# Autodesk Inventor assembly: Tamiya SRB u joint
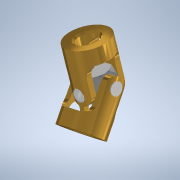
[picture p0: Inventor's stored thumbnail of the model, 180x180]
Saved by Autodesk Inventor 2020 (Build 240168000, 168)
## iProperties
Created: 2015-10-12
Part Number: Tamiya SRB u joint
Document SubType Name: Assembly
Designer: Vikki
Sending System: SolidWorks 2015
Last Author: Tompkins
Last Saved: 2015-10-12
Author: Vikki
## Documents named in this file (12)
- D:\borewell rescuebot\pll manipulator files\sps manipulator\Tamiya SRB u joint.iam
- D:\borewell rescuebot\pll manipulator files\sps manipulator\center block u joint.ipt
- D:\borewell rescuebot\pll manipulator files\sps manipulator\Tamiya u joint.ipt
- D:\borewell rescuebot\pll manipulator files\sps manipulator\large pin.ipt
- D:\borewell rescuebot\pll manipulator files\sps manipulator\small rivit.ipt
- D:\borewell rescuebot\pll manipulator files\sps manipulator\Tamiya u joint - 2.ipt
- D:\borewell rescuebot\pll manipulator files\sps manipulator\Tamiya SRB u joint\AIP\FEA\dh3epo728.fins
- D:\borewell rescuebot\pll manipulator files\sps manipulator\Tamiya SRB u joint\AIP\FEA\dh3epo728.fsat
- D:\borewell rescuebot\pll manipulator files\sps manipulator\Tamiya SRB u joint\AIP\FEA\dh3epo728.ftes
- D:\borewell rescuebot\pll manipulator files\sps manipulator\Tamiya SRB u joint\AIP\FEA\dh3epo728.fwiz
- D:\borewell rescuebot\pll manipulator files\sps manipulator\Tamiya SRB u joint\AIP\FEA\dh3epo734.fmsh
- D:\borewell rescuebot\pll manipulator files\sps manipulator\Tamiya SRB u joint\AIP\FEA\dh3epo735.fres
## Components (5 placed, 5 different names)
1. center block u joint:1 — Mate:3, Mate:4, Mate:7, Mate:11, Mate:12
2. Tamiya u joint:1 — Mate:7, Mate:11, Flush:1
3. large pin:1 — Mate:3, Mate:4, Mate:5, Mate:10
4. small rivit:1 — Mate:5, Flush:1
5. Tamiya u joint - 2:1 — Mate:10, Mate:12
## Relationships (8: Mate 7, Flush 1)
- Mate:3: center block u joint:1 ↔ large pin:1
- Mate:4: center block u joint:1 ↔ large pin:1
- Mate:5: large pin:1 ↔ small rivit:1
- Mate:7: center block u joint:1 ↔ Tamiya u joint:1
- Mate:10: large pin:1 ↔ Tamiya u joint - 2:1
- Mate:11 (0.165 mm): center block u joint:1 ↔ Tamiya u joint:1
- Flush:1 (2.4 mm): Tamiya u joint:1 ↔ small rivit:1
- Mate:12 (0.1615 mm): center block u joint:1 ↔ Tamiya u joint - 2:1
## Named parameters: sa_0 = 2940, sa_2 = 3000
note: some values were not read from the file. Shown as the stored number, unit unknown: "sa_0", "sa_2".
